# Autodesk Inventor assembly: Chassis assembly
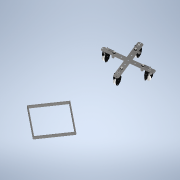
[picture p0: Inventor's stored thumbnail of the model, 180x180]
Saved by Autodesk Inventor 2020 (Build 240168000, 168)
## iProperties
Created: 2022-07-02
Part Number: Chassis assembly
Document SubType Name: Assembly
Designer: karimi2
Author: karimi2
## Documents named in this file (3)
- C:\Users\karimi2\Documents\PROJECT\src\Chassis assembly.iam
- C:\Users\karimi2\Documents\PROJECT\src\Chassis base shaft.ipt
- C:\Users\karimi2\Documents\PROJECT\src\Chassis and wheels assembly.iam
## Components (5 placed, 2 different names)
1. Chassis base shaft:1 — Rigid:3
2. Chassis base shaft:2 — Rigid:4
3. Chassis base shaft:3 — Rigid:2, Rigid:3
4. Chassis base shaft:4 — Rigid:2, Rigid:4
5. Chassis and wheels assembly:1 [sub-assembly]
## Relationships (3: WeldJoint 3)
- Rigid:2 [WeldJoint]: Chassis base shaft:3 ↔ Chassis base shaft:4
- Rigid:3 [WeldJoint]: Chassis base shaft:1 ↔ Chassis base shaft:3
- Rigid:4 [WeldJoint]: Chassis base shaft:2 ↔ Chassis base shaft:4
